# Autodesk Inventor assembly: Dual Omni Wheel
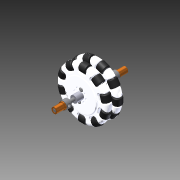
[picture p0: Inventor's stored thumbnail of the model, 180x180]
Saved by Autodesk Inventor 2015 (Build 190159000, 159)
## iProperties
Created: 2014-10-15
Part Number: Dual Omni Wheel
Document SubType Name: Assembly
Designer: lethcoec
Author: lethcoec
## Documents named in this file (8)
- \\st-svr\studenthdrives$\18\LethcoeC\FTC Cascade effect\FTC Parts\Subassemblies\Dual Omni Wheel.iam
- \\st-svr\studenthdrives$\18\LethcoeC\FTC Cascade effect\Imported Components\AxleHub1\AxleHub1.ipt
- \\st-svr\studenthdrives$\18\LethcoeC\FTC Cascade effect\3inch OmniWheel.iam
- \\st-svr\studenthdrives$\18\LethcoeC\FTC Cascade effect\Imported Components\Screw5\Screw5.ipt
- \\st-svr\studenthdrives$\18\LethcoeC\FTC Cascade effect\Imported Components\Axle100mm\Axle100mm.ipt
- \\st-svr\studenthdrives$\18\LethcoeC\FTC Cascade effect\FTC Parts\Subassemblies\Spacer.ipt
- \\st-svr\studenthdrives$\18\LethcoeC\FTC Cascade effect\FTC Parts\Subassemblies\Axle hub with no cricle thing.ipt
- \\st-svr\studenthdrives$\18\LethcoeC\FTC Cascade effect\FTC Parts\Subassemblies\Bushing.ipt
## Components (14 placed, 7 different names)
1. AxleHub1:1 — Mate:1, Mate:2, Mate:3, Mate:4
2. 3inch OmniWheel:1 [sub-assembly] — Mate:3, Mate:4, Mate:7, Mate:8, Mate:13, Mate:14, Mate:15, Mate:22
3. 3inch OmniWheel:2 [sub-assembly] — Mate:1, Mate:2, Mate:9, Mate:10, Mate:11, Mate:12, Mate:25
4. Screw5:2 — Mate:7, Mate:8
5. Screw5:3 — Mate:9, Mate:10
6. Screw5:4 — Mate:11, Mate:12
7. Screw5:5 — Mate:13, Mate:14
8. Axle100mm:1 — Mate:15, Mate:16, Mate:17, Mate:18, Mate:19, Mate:28, Mate:30
9. Spacer:3 — Mate:16, Mate:22
10. Spacer:4 — Mate:17, Mate:25
11. Axle hub with no cricle thing:1 — Mate:19, Mate:31
12. Axle hub with no cricle thing:2 — Mate:18, Mate:29
13. Bushing:1 — Mate:28, Mate:29
14. Bushing:2 — Mate:30, Mate:31
## Relationships (23: Mate 23)
- Mate:1: AxleHub1:1 ↔ 3inch OmniWheel:2
- Mate:2: AxleHub1:1 ↔ 3inch OmniWheel:2
- Mate:3: AxleHub1:1 ↔ 3inch OmniWheel:1
- Mate:4: AxleHub1:1 ↔ 3inch OmniWheel:1
- Mate:7: 3inch OmniWheel:1 ↔ Screw5:2
- Mate:8: 3inch OmniWheel:1 ↔ Screw5:2
- Mate:9: 3inch OmniWheel:2 ↔ Screw5:3
- Mate:10: 3inch OmniWheel:2 ↔ Screw5:3
- Mate:11: 3inch OmniWheel:2 ↔ Screw5:4
- Mate:12: 3inch OmniWheel:2 ↔ Screw5:4
- Mate:13: 3inch OmniWheel:1 ↔ Screw5:5
- Mate:14: 3inch OmniWheel:1 ↔ Screw5:5
- Mate:15: 3inch OmniWheel:1 ↔ Axle100mm:1
- Mate:16: Axle100mm:1 ↔ Spacer:3
- Mate:17: Axle100mm:1 ↔ Spacer:4
- Mate:18: Axle100mm:1 ↔ Axle hub with no cricle thing:2
- Mate:19: Axle100mm:1 ↔ Axle hub with no cricle thing:1
- Mate:22: 3inch OmniWheel:1 ↔ Spacer:3
- Mate:25: 3inch OmniWheel:2 ↔ Spacer:4
- Mate:28: Axle100mm:1 ↔ Bushing:1
- Mate:29: Axle hub with no cricle thing:2 ↔ Bushing:1
- Mate:30: Axle100mm:1 ↔ Bushing:2
- Mate:31: Axle hub with no cricle thing:1 ↔ Bushing:2
